# Autodesk Inventor assembly: Fixture Assembly
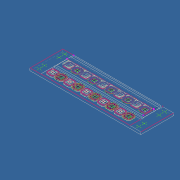
[picture p0: Inventor's stored thumbnail of the model, 180x180]
Saved by Autodesk Inventor 2016 (Build 200138000, 138)
## iProperties
Created: 2016-04-08
Part Number: Fixture Assembly
Document SubType Name: Assembly
Designer: Sam Clay
Author: Sam Clay
## Documents named in this file (4)
- Z:\enclosure\inventor\Fixture Assembly.iam
- Z:\enclosure\inventor\Fixture Base.ipt
- Z:\enclosure\inventor\Case Top.ipt
- Z:\enclosure\inventor\Case Bottom.ipt
## Components (21 placed, 3 different names)
1. Fixture Base:1 — Planar:5, Planar:6, Planar:7, Mate:4, Mate:5, Mate:6
2. Case Bottom:1 — Planar:6, Mate:6, Mate:7
3. Case Bottom:2
4. Case Bottom:3
5. Case Bottom:4
6. Case Bottom:5
7. Case Top:2 — Planar:7, Mate:4, Mate:5, Mate:7
8. Case Top:3
9. Case Top:4
10. Case Top:5
11. Case Top:6
12. Case Top:1 — Mate:2, Mate:3
13. Case Top:7
14. Case Top:8
15. Case Top:9
16. Case Top:10
17. Case Bottom:6 — Planar:5, Mate:2, Mate:3
18. Case Bottom:7
19. Case Bottom:8
20. Case Bottom:9
21. Case Bottom:10
## Component patterns: (5 elements, first: Case Bottom:1), (5 elements, first: Case Top:2), (5 elements, first: Case Top:1), (5 elements, first: Case Bottom:6)
## Relationships (9: Mate 6, PlanarJoint 3)
- Planar:5 (16.51 mm): Fixture Base:1 ↔ Case Bottom:6
- Planar:6: Fixture Base:1 ↔ Case Bottom:1
- Mate:2 (6.604 mm): Case Top:1 ↔ Case Bottom:6
- Mate:3: Case Top:1 ↔ Case Bottom:6
- Planar:7: Fixture Base:1 ↔ Case Top:2
- Mate:4 (6.604 mm): Fixture Base:1 ↔ Case Top:2
- Mate:5 (6.604 mm): Fixture Base:1 ↔ Case Top:2
- Mate:6 (6.604 mm): Fixture Base:1 ↔ Case Bottom:1
- Mate:7 (6.604 mm): Case Bottom:1 ↔ Case Top:2
